# Autodesk Inventor assembly: Buffer_L
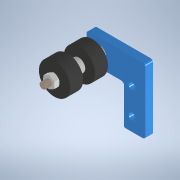
[picture p0: Inventor's stored thumbnail of the model, 180x180]
Saved by Autodesk Inventor 2021 (Build 250183000, 183)
## iProperties
Created: 2021-09-25
Part Number: Buffer_L
Document SubType Name: Assembly
Designer: Jorian Brusind
Author: Jorian Brusind
## Documents named in this file (7)
- C:\Users\Jorian Brusind\Documents\GitHub\HyperRail\Inventor Files\Buffer_L.iam
- C:\Users\Jorian Brusind\Documents\GitHub\HyperRail\Inventor Files\Buffer_Mount.ipt
- C:\Users\Jorian Brusind\Documents\GitHub\HyperRail\Inventor Files\11mm_BearingWheel.ipt
- C:\Users\Jorian Brusind\Documents\GitHub\HyperRail\Inventor Files\Metric bolt\Bolt M5 50mm.ipt
- C:\Users\Jorian Brusind\Documents\GitHub\HyperRail\Inventor Files\5mm_Spacer.ipt
- C:\Users\Jorian Brusind\Documents\GitHub\HyperRail\Inventor Files\8mm_Spacer.ipt
- C:\Users\Jorian Brusind\Documents\GitHub\PersonalProjects\HyperRail\Inventor Files\Metric nuts\Nut M5.ipt
## Components (7 placed, 6 different names)
1. 11mm_BearingWheel:1 — Mate:8, Mate:15, Mate:22
2. 11mm_BearingWheel:2 — Mate:9, Mate:13, Mate:18
3. Bolt M5 50mm:1 — Mate:8, Mate:9, Mate:11, Mate:12, Mate:19, Mate:20, Mate:21
4. 5mm_Spacer:1 — Mate:11, Mate:17, Mate:18
5. 8mm_Spacer:1 — Mate:12, Mate:13, Mate:15
6. Buffer_Mount:1 — Mate:17, Mate:19, Mate:20
7. Nut M5:1 — Mate:21, Mate:22
## Relationships (12: Mate 12)
- Mate:8: 11mm_BearingWheel:1 ↔ Bolt M5 50mm:1
- Mate:9: 11mm_BearingWheel:2 ↔ Bolt M5 50mm:1
- Mate:11: Bolt M5 50mm:1 ↔ 5mm_Spacer:1
- Mate:12: Bolt M5 50mm:1 ↔ 8mm_Spacer:1
- Mate:13: 11mm_BearingWheel:2 ↔ 8mm_Spacer:1
- Mate:15: 11mm_BearingWheel:1 ↔ 8mm_Spacer:1
- Mate:17: 5mm_Spacer:1 ↔ Buffer_Mount:1
- Mate:18: 11mm_BearingWheel:2 ↔ 5mm_Spacer:1
- Mate:19: Bolt M5 50mm:1 ↔ Buffer_Mount:1
- Mate:20: Bolt M5 50mm:1 ↔ Buffer_Mount:1
- Mate:21: Bolt M5 50mm:1 ↔ Nut M5:1
- Mate:22: 11mm_BearingWheel:1 ↔ Nut M5:1
